# Autodesk Inventor assembly: opencm9_grp
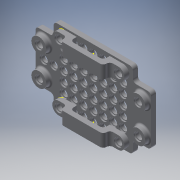
[picture p0: Inventor's stored thumbnail of the model, 180x180]
Saved by Autodesk Inventor 2016 (Build 200138000, 138)
## iProperties
Created: 2016-02-15
Part Number: opencm9_grp
Document SubType Name: Assembly
Designer: jforce
Author: jforce
## Documents named in this file (3)
- C:\Users\jforce\Dropbox\gmu\ece590 (Selective Sync Conflict)\models3\opencm9_grp.iam
- C:\Users\jforce\Dropbox\gmu\ece590 (Selective Sync Conflict)\models3\opencm_strap.ipt
- C:\Users\jforce\Dropbox\gmu\ece590 (Selective Sync Conflict)\models3\opencm9_mount.ipt
## Components (3 placed, 2 different names)
1. opencm_strap:1 — Mate:2, Mate:3
2. opencm9_mount:1 — Mate:1, Mate:2, Mate:3, Mate:4
3. opencm_strap:2 — Mate:1, Mate:4
## Relationships (4: Mate 4)
- Mate:1: opencm9_mount:1 ↔ opencm_strap:2
- Mate:2: opencm_strap:1 ↔ opencm9_mount:1
- Mate:3: opencm_strap:1 ↔ opencm9_mount:1
- Mate:4: opencm9_mount:1 ↔ opencm_strap:2
